# Autodesk Inventor assembly: Version 2 mockup
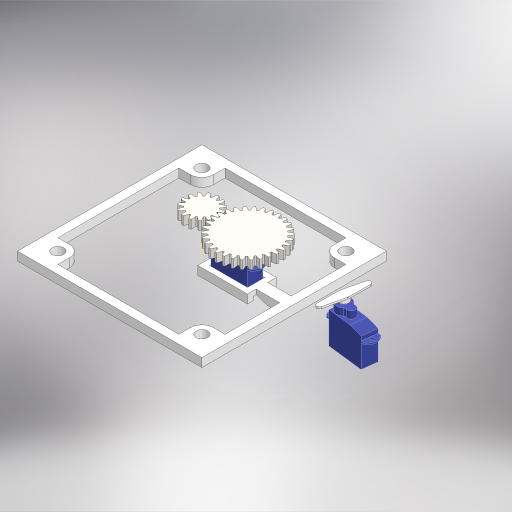
[picture p0: Inventor's stored thumbnail of the model, 512x512]
Saved by Autodesk Inventor 2024 (Build 280153000, 153)
## iProperties
Created: 2023-10-08
Part Number: Version 2 mockup
Document SubType Name: Assembly
Designer: byrne
Author: byrne
## Documents named in this file (5)
- C:\Users\byrne\OneDrive\Documents\Inventor\RAI\Version 2 mockup.iam
- C:\Users\byrne\OneDrive\Documents\Inventor\RAI\Pololu#1053 v4.ipt
- C:\Users\byrne\OneDrive\Documents\Inventor\RAI\Dual Servo Attachment.ipt
- C:\Users\byrne\OneDrive\Documents\Inventor\RAI\footprint.ipt
- C:\Users\byrne\OneDrive\Documents\Inventor\RAI\Version 2 mockup\Design Accelerator\Spur Gears1.iam
## Components (6 placed, 4 different names)
1. footprint:1 — Mate:6, Mate:7, Flush:1, Mate:10
2. Pololu#1053 v4:1 — Insert:1, Mate:6, Mate:7, Flush:1, Mate:8, Mate:9, Mate:11
3. Pololu#1053 v4:2 — Insert:4
4. Dual Servo Attachment:1 — Insert:1
5. Dual Servo Attachment:2 — Insert:4
6. Spur Gears:1 [sub-assembly] — Mate:8, Mate:9, Mate:10, Mate:11
## Relationships (9: Mate 6, Insert 2, Flush 1)
- Insert:1: Pololu#1053 v4:1 ↔ Dual Servo Attachment:1
- Insert:4: Pololu#1053 v4:2 ↔ Dual Servo Attachment:2
- Mate:6 (0.5 mm): footprint:1 ↔ Pololu#1053 v4:1
- Mate:7 (0.5 mm): footprint:1 ↔ Pololu#1053 v4:1
- Flush:1: footprint:1 ↔ Pololu#1053 v4:1
- Mate:8: Pololu#1053 v4:1 ↔ Spur Gears:1
- Mate:9: Pololu#1053 v4:1 ↔ Spur Gears:1
- Mate:10: footprint:1 ↔ Spur Gears:1
- Mate:11: Pololu#1053 v4:1 ↔ Spur Gears:1
